# Autodesk Inventor assembly: frame assy
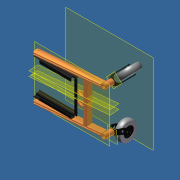
[picture p0: Inventor's stored thumbnail of the model, 180x180]
Saved by Autodesk Inventor 2012 (Build 160160000, 160)
## iProperties
Created: 2012-03-07
Part Number: frame assy
Document SubType Name: Assembly
Designer: esv
Mass: 22101.3 g
Surface Area: 8904.59 cm^2
Volume: 6785.47 cm^3
Density: 3.25715 g/cm^3
Author: esv
## Documents named in this file (4)
- C:\Users\Ed\Documents\masters\CAD\Invacare\frame assy.iam
- C:\Users\Ed\Documents\masters\CAD\Invacare\caster assy.iam
- C:\Users\Ed\Documents\masters\CAD\Invacare\frame.ipt
- C:\Users\Ed\Documents\masters\CAD\Invacare\battery rails.ipt
## Components (4 placed, 3 different names)
1. caster assy:1 [sub-assembly] — Insert:1
2. caster assy:2 [sub-assembly] — Insert:2
3. frame:1 — Insert:1, Insert:2, Angle:2, Mate:9, Flush:10, Angle:3
4. battery rails:1 — Mate:7, Flush:3, Mate:9, Flush:10
## Relationships (8: Insert 2, Mate 2, Flush 2, Angle 2)
- Insert:1: caster assy:1 ↔ frame:1
- Insert:2: caster assy:2 ↔ frame:1
- Mate:7: battery rails:1
- Flush:3: battery rails:1
- Angle:2 (0 deg): frame:1
- Mate:9: frame:1 ↔ battery rails:1
- Flush:10: frame:1 ↔ battery rails:1
- Angle:3 (0 deg): frame:1
